# Autodesk Inventor assembly: TelescopingArmSpringDriven_MIR
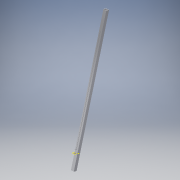
[picture p0: Inventor's stored thumbnail of the model, 180x180]
Saved by Autodesk Inventor 2016 SP1 (Build 200210100, 210)
## iProperties
Created: 2016-01-26
Part Number: TelescopingArmSpringDriven_MIR
Document SubType Name: Assembly
Designer: steele
Author: steele
## Documents named in this file (3)
- C:\snobotics\CAD-Development\robSteele\SnoBotics2016\2016-01-31-Lift\TelescopingArmSpringDriven_MIR.iam
- C:\snobotics\CAD-Development\robSteele\SnoBotics2016\TelescopeArm\OuterTube_MIR.ipt
- C:\snobotics\CAD-Development\robSteele\SnoBotics2016\TelescopeArm\InnerTube_MIR.ipt
## Components (2 placed, 2 different names)
1. OuterTube_MIR:1 — Flush:2, Mate:4, Mate:3
2. InnerTube_MIR:1 — Flush:2, Mate:4, Mate:3
## Relationships (3: Mate 2, Flush 1)
- Flush:2 (-127 mm): OuterTube_MIR:1 ↔ InnerTube_MIR:1
- Mate:4: OuterTube_MIR:1 ↔ InnerTube_MIR:1
- Mate:3: OuterTube_MIR:1 ↔ InnerTube_MIR:1
